# Autodesk Inventor assembly: Hopper Rest 8-32
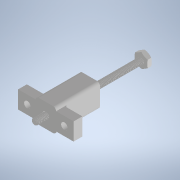
[picture p0: Inventor's stored thumbnail of the model, 180x180]
Saved by Autodesk Inventor 2022.1 (Build 261234000, 234)
## iProperties
Created: 2021-06-04
Part Number: Hopper Rest 8-32
Document SubType Name: Assembly
Designer: John
Author: John
## Documents named in this file (4)
- C:\Users\owner\Desktop\Project 3 Modelling\Project 3 Autodesk Inventor Files\6. Misc Parts\1. Resting Block\Hopper Rest 8-32.iam
- C:\Users\owner\Desktop\Project 3 Modelling\Project 3 Autodesk Inventor Files\6. Misc Parts\1. Resting Block\Hopper Rest Metric Wide.ipt
- C:\Users\owner\Desktop\Project 3 Modelling\Project 3 Autodesk Inventor Files\6. Misc Parts\1. Resting Block\8-32 x 3 Inch Threaded Rod.ipt
- C:\Users\owner\Desktop\Project 3 Modelling\Project 3 Autodesk Inventor Files\6. Misc Parts\1. Resting Block\8-32 Hex Nut.ipt
## Components (4 placed, 3 different names)
1. Hopper Rest Metric Wide:1 — Angle:1, Mate:1, Mate:2, Mate:4
2. 8-32 x 3 Inch Threaded Rod:1 — Mate:3, Flush:1, Mate:4, Insert:1, Rotation:1
3. 8-32 Hex Nut:1 — Angle:1, Mate:1, Mate:2, Insert:1
4. 8-32 Hex Nut:2 — Mate:3, Flush:1, Rotation:1
## Relationships (8: Mate 4, Angle 1, Flush 1, Insert 1, RelateRotation 1)
- Angle:1 (0 deg): Hopper Rest Metric Wide:1 ↔ 8-32 Hex Nut:1
- Mate:1: Hopper Rest Metric Wide:1 ↔ 8-32 Hex Nut:1
- Mate:2: Hopper Rest Metric Wide:1 ↔ 8-32 Hex Nut:1
- Mate:3: 8-32 x 3 Inch Threaded Rod:1 ↔ 8-32 Hex Nut:2
- Flush:1: 8-32 x 3 Inch Threaded Rod:1 ↔ 8-32 Hex Nut:2
- Mate:4: Hopper Rest Metric Wide:1 ↔ 8-32 x 3 Inch Threaded Rod:1
- Insert:1 (-37.8973 mm): 8-32 x 3 Inch Threaded Rod:1 ↔ 8-32 Hex Nut:1
- Rotation:1 [RelateRotation] (1 ul): 8-32 x 3 Inch Threaded Rod:1 ↔ 8-32 Hex Nut:2
